# Autodesk Inventor assembly: #Spindexer
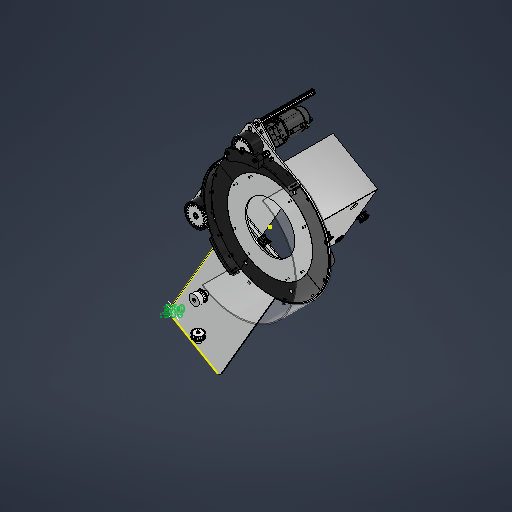
[picture p0: Inventor's stored thumbnail of the model, 512x512]
Saved by Autodesk Inventor 2026 (Build 300175000, 175)
## iProperties
Created: 2026-02-05
Part Number: #Spindexer
Document SubType Name: Assembly
Designer: Owen L
Mass: 7910.07 g
Surface Area: 22164.7 cm^2
Volume: 5901.9 cm^3
Density: 1.34026 g/cm^3
Author: Owen L
## Documents named in this file (54)
- C:\Users\littl\OneDrive\Documents\GitHub\2026-Robot-Mechanical\Spindexer\#Spindexer.iam
- C:\Users\littl\OneDrive\Documents\GitHub\2026-Robot-Mechanical\Spindexer\3DPRINT,KICKER,RAMP.ipt
- C:\Users\littl\OneDrive\Documents\GitHub\2026-Robot-Mechanical\#1_CAD Library\Power Transmission\Bearings\PURCHASED,HEX_BEARING.ipt
- C:\Users\littl\OneDrive\Documents\GitHub\2026-Robot-Mechanical\#1_CAD Library\Building Materials\Fasteners\Bolts\PURCHASED,10-32x0.5in,BUTTONHEAD,BOLT.ipt
- C:\Users\littl\OneDrive\Documents\GitHub\2026-Robot-Mechanical\#1_CAD Library\Building Materials\Fasteners\Nuts\PURCHASED,NYLOCK,10-32,NUT.ipt
- C:\Users\littl\OneDrive\Documents\GitHub\2026-Robot-Mechanical\#1_CAD Library\Building Materials\Fasteners\Bolts\PURCHASED,10-32x0.625in,BUTTONHEAD,BOLT.ipt
- C:\Users\littl\OneDrive\Documents\GitHub\2026-Robot-Mechanical\Spindexer\PLATE,SHOOTER,MOUNT.ipt
- C:\Users\littl\OneDrive\Documents\GitHub\2026-Robot-Mechanical\Spindexer\PLATE,TURRET,ENCODER,GEAR.ipt
- C:\Users\littl\OneDrive\Documents\GitHub\2026-Robot-Mechanical\Spindexer\PLATE,TURRET,PINNION,GEAR.ipt
- C:\Users\littl\OneDrive\Documents\GitHub\2026-Robot-Mechanical\Spindexer\PLATE,TURRET,MOTOR,MOUNT.ipt
- C:\Users\littl\OneDrive\Documents\GitHub\2026-Robot-Mechanical\#1_CAD Library\Electronics\CONTROLS,ENCODER,HEX_BORE.ipt
- C:\Users\littl\OneDrive\Documents\GitHub\2026-Robot-Mechanical\Spindexer\STOCK,HEX,SHAFT,TURRET,DRIVE.ipt
- C:\Users\littl\OneDrive\Documents\GitHub\2026-Robot-Mechanical\Spindexer\STOCK,HEX,SHAFT,TURRET,ENCODER.ipt
- C:\Users\littl\OneDrive\Documents\GitHub\2026-Robot-Mechanical\Spindexer\3DPRINT,TURRET,HEX,SPACER.ipt
- C:\Users\littl\OneDrive\Documents\GitHub\2026-Robot-Mechanical\Spindexer\STOCK,CHURRO,HEX,TURRET,MOTOR-MOUNT,SPACER.ipt
- C:\Users\littl\OneDrive\Documents\GitHub\2026-Robot-Mechanical\#1_CAD Library\Building Materials\Fasteners\Bolts\PURCHASED,0.25-20x0.5in,BUTTONHEAD,BOLT.ipt
- C:\Users\littl\OneDrive\Documents\GitHub\2026-Robot-Mechanical\Spindexer\MOTOR,VEX,FALCON,500.ipt
- C:\Users\littl\OneDrive\Documents\GitHub\2026-Robot-Mechanical\#1_CAD Library\Power Transmission\MaxPlanetary\PURCHASED,REV,MAX-PLANETARY,SINGLE-STAGE,FALCON-TO-HEX.ipt
- C:\Users\littl\OneDrive\Documents\GitHub\2026-Robot-Mechanical\#1_CAD Library\Building Materials\Fasteners\Washers\PURCHASED,WASHER,10-32.ipt
- C:\Users\littl\OneDrive\Documents\GitHub\2026-Robot-Mechanical\Spindexer\3DPRINT,CABLE-SHROUD,QUARTER.ipt
- C:\Users\littl\OneDrive\Documents\GitHub\2026-Robot-Mechanical\Spindexer\3DPRINT,CABLE,TRAY,BL.ipt
- C:\Users\littl\OneDrive\Documents\GitHub\2026-Robot-Mechanical\Spindexer\3DPRINT,CABLE,TRAY,BR.ipt
- C:\Users\littl\OneDrive\Documents\GitHub\2026-Robot-Mechanical\Spindexer\3DPRINT,CABLE,TRAY,TL.ipt
- C:\Users\littl\OneDrive\Documents\GitHub\2026-Robot-Mechanical\Spindexer\3DPRINT,CABLE,TRAY,TR.ipt
- C:\Users\littl\OneDrive\Documents\GitHub\2026-Robot-Mechanical\Spindexer\PLATE,SHOOTER,SHEILD,LOWER.ipt
- C:\Users\littl\OneDrive\Documents\GitHub\2026-Robot-Mechanical\Spindexer\3DPRINT,TURRET,PINION,SHROUD.ipt
- C:\Users\littl\OneDrive\Documents\GitHub\2026-Robot-Mechanical\#1_CAD Library\Building Materials\Fasteners\Bolts\PURCHASED,10-32x0.75in,BUTTONHEAD,BOLT.ipt
- C:\Users\littl\OneDrive\Documents\GitHub\2026-Robot-Mechanical\Spindexer\3DPRINT,TURRET,PINION,SHROUD,21T.ipt
- C:\Users\littl\OneDrive\Documents\GitHub\2026-Robot-Mechanical\Spindexer\STOCK,CHURRO,HEX,TURRET,MOTOR-MOUNT,SUPPORT.ipt
- C:\Users\littl\OneDrive\Documents\GitHub\2026-Robot-Mechanical\Spindexer\3DPRINT,TURRET,LOCK.ipt
- C:\Users\littl\OneDrive\Documents\GitHub\2026-Robot-Mechanical\Spindexer\STOCK,CHURRO,HEX,TURRET,LOCK.ipt
- C:\Users\littl\OneDrive\Documents\GitHub\2026-Robot-Mechanical\#1_CAD Library\Building Materials\Fasteners\Bolts\PURCHASED,0.25-20x0.875in,SOCKETHEAD,BOLT.ipt
- C:\Users\littl\OneDrive\Documents\GitHub\2026-Robot-Mechanical\Spindexer\PLATE,BACK.ipt
- C:\Users\littl\OneDrive\Documents\GitHub\2026-Robot-Mechanical\Spindexer\PLATE,FRONT.ipt
- C:\Users\littl\OneDrive\Documents\GitHub\2026-Robot-Mechanical\Spindexer\WCP-0564.ipt
- C:\Users\littl\OneDrive\Documents\GitHub\2026-Robot-Mechanical\#1_CAD Library\Wheels\Compliant\PURCHASED,WHEEL,COMPLIANT,2.25in.ipt
- C:\Users\littl\OneDrive\Documents\GitHub\2026-Robot-Mechanical\Spindexer\PLATE,BEARING,BLOCK.ipt
- C:\Users\littl\OneDrive\Documents\GitHub\2026-Robot-Mechanical\Spindexer\PLATE,BEARING,BLOCK,TOP.ipt
- C:\Users\littl\OneDrive\Documents\GitHub\2026-Robot-Mechanical\Spindexer\Kicker.ipt
- C:\Users\littl\OneDrive\Documents\GitHub\2026-Robot-Mechanical\#1_CAD Library\Motors\MOTOR,NEO,V2.0.ipt
- C:\Users\littl\OneDrive\Documents\GitHub\2026-Robot-Mechanical\Spindexer\PLATE_LEFT.ipt
- C:\Users\littl\OneDrive\Documents\GitHub\2026-Robot-Mechanical\Spindexer\PLATE,BELT,REVERSER.ipt
- C:\Users\littl\OneDrive\Documents\GitHub\2026-Robot-Mechanical\Spindexer\WCP-0562.ipt
- C:\Users\littl\OneDrive\Documents\GitHub\2026-Robot-Mechanical\Spindexer\REV-21-1921.ipt
- C:\Users\littl\OneDrive\Documents\GitHub\2026-Robot-Mechanical\Spindexer\WCP-2057.ipt
- C:\Users\littl\OneDrive\Documents\GitHub\2026-Robot-Mechanical\Spindexer\WCP-1420.ipt
- C:\Users\littl\OneDrive\Documents\GitHub\2026-Robot-Mechanical\Spindexer\STOCK,LEFT,HEX.ipt
- C:\Users\littl\OneDrive\Documents\GitHub\2026-Robot-Mechanical\Spindexer\STOCK,REVERSER,HEX.ipt
- C:\Users\littl\OneDrive\Documents\GitHub\2026-Robot-Mechanical\Spindexer\STOCK,TOP-RIGHT,HEX.ipt
- C:\Users\littl\OneDrive\Documents\GitHub\2026-Robot-Mechanical\Spindexer\STOCK,BOTTOM-RIGHT,HEX.ipt
- C:\Users\littl\OneDrive\Documents\GitHub\2026-Robot-Mechanical\Spindexer\3DPRINT,ROLLER,PLUG,SHORT.ipt
- C:\Users\littl\OneDrive\Documents\GitHub\2026-Robot-Mechanical\Spindexer\3DPRINT,ROLLER,PLUG,LONG.ipt
- C:\Users\littl\OneDrive\Documents\GitHub\2026-Robot-Mechanical\Spindexer\STOCK,KICKER,HEX.ipt
- C:\Users\littl\OneDrive\Documents\GitHub\2026-Robot-Mechanical\Spindexer\3DPRINT,VERTICAL,ROLLER,TOP,BEARING,BLOCK.ipt
## Components (129 placed, 53 different names)
1. 3DPRINT,VERTICAL,ROLLER,TOP,BEARING,BLOCK:1 — Mate:309, Insert:317
2. 3DPRINT,TURRET,PINION,SHROUD:1 — Mate:224, Mate:225, Mate:226, Insert:267
3. PURCHASED,10-32x0.75in,BUTTONHEAD,BOLT:1 — Insert:268, Mate:232
4. PURCHASED,10-32x0.75in,BUTTONHEAD,BOLT:2 — Insert:267, Mate:236
5. 3DPRINT,TURRET,PINION,SHROUD,21T:1 — Mate:227, Mate:228, Mate:229, Insert:268
6. STOCK,CHURRO,HEX,TURRET,MOTOR-MOUNT,SPACER:7 — Insert:272
7. STOCK,CHURRO,HEX,TURRET,MOTOR-MOUNT,SPACER:8 — Insert:273
8. PURCHASED,0.25-20x0.5in,BUTTONHEAD,BOLT:16 — Insert:279
9. PURCHASED,0.25-20x0.5in,BUTTONHEAD,BOLT:17 — Insert:280
10. PURCHASED,0.25-20x0.5in,BUTTONHEAD,BOLT:18 — Insert:281
11. STOCK,CHURRO,HEX,TURRET,MOTOR-MOUNT,SUPPORT:1 — Insert:282
12. 3DPRINT,TURRET,LOCK:1 — Mate:237, Mate:238, Flush:35, Insert:285, Insert:286
13. STOCK,CHURRO,HEX,TURRET,LOCK:1 — Insert:283
14. STOCK,CHURRO,HEX,TURRET,LOCK:2 — Insert:284
15. PURCHASED,0.25-20x0.875in,SOCKETHEAD,BOLT:1 — Insert:285
16. PURCHASED,0.25-20x0.875in,SOCKETHEAD,BOLT:2 — Insert:286
17. PURCHASED,0.25-20x0.5in,BUTTONHEAD,BOLT:19 — Insert:287
18. PURCHASED,0.25-20x0.5in,BUTTONHEAD,BOLT:20 — Insert:288
19. PLATE,BACK:1 — Mate:240, Mate:264, Flush:44, Mate:267, Flush:48, Flush:52, Mate:277, Mate:278, Mate:280, Insert:305, Insert:306, Insert:309, Insert:312, Insert:314, Insert:316, Mate:269
20. PLATE,FRONT:1 — Mate:264, Flush:44, Mate:265, Mate:268, Mate:270, Insert:303, Flush:49, Mate:274, Flush:51, Insert:311, Insert:313, Insert:315, Mate:306, Mate:311
21. WCP-0564:1 — Mate:267, Mate:298, Flush:64, Flush:66
22. PURCHASED,WHEEL,COMPLIANT,2.25in:1 — Mate:268, Mate:269, Insert:298, Mate:270
23. PURCHASED,WHEEL,COMPLIANT,2.25in:3 — Insert:298, Mate:309
24. PLATE,BEARING,BLOCK:1 — Flush:48, Flush:53, Insert:308
25. PLATE,BEARING,BLOCK,TOP:1 — Mate:272, Mate:278, Flush:53, Insert:310
26. KICKER_GEARBOX — Insert:303, Flush:49, Insert:304, Flush:50
27. MOTOR,NEO,V2.0:1 — Insert:304, Flush:50
28. PLATE_LEFT:1 — Mate:274, Flush:51, Mate:275
29. PLATE,BELT,REVERSER:1 — Mate:280, Insert:307
30. WCP-0562:1 — Mate:285, Flush:56, Flush:58
31. REV-21-1921:1 — Mate:282, Flush:54
32. REV-21-1921:2 — Mate:281, Flush:54, Mate:290, Mate:291
33. WCP-2057:1 — Insert:308, Mate:287, Flush:59
34. WCP-2057:2 — Insert:307, Mate:283, Mate:291, Flush:60
35. WCP-2057:3 — Insert:306, Mate:282, Mate:287, Mate:292, Mate:296
36. WCP-2057:4 — Insert:305, Mate:281, Mate:288, Mate:289, Mate:297
37. WCP-2057:5 — Insert:311, Flush:62
38. WCP-2057:6 — Insert:310, Mate:286, Flush:61
39. WCP-2057:7 — Insert:313, Flush:63
40. WCP-2057:8 — Insert:309, Mate:284, Mate:285, Mate:286, Mate:295
41. WCP-2057:9 — Insert:312, Mate:293, Mate:299, Mate:312
42. WCP-2057:11 — Insert:314, Mate:294, Mate:300
43. WCP-2057:12 — Insert:316, Mate:298
44. WCP-2057:13 — Insert:315, Mate:301, Mate:302, Mate:305
45. WCP-1420:1 — Mate:283, Mate:288, Flush:55, Mate:289, Mate:290
46. WCP-1420:2 — Mate:284, Flush:55
47. WCP-0562:2 — Mate:292, Flush:56
48. WCP-0562:3 — Mate:293, Flush:57, Flush:58
49. WCP-0562:4 — Mate:294, Flush:57
50. STOCK,LEFT,HEX:1 — Mate:295, Flush:61
51. STOCK,LEFT,HEX:2 — Mate:296, Flush:59
52. STOCK,REVERSER,HEX:1 — Mate:297, Flush:60
53. STOCK,TOP-RIGHT,HEX:1 — Mate:299, Flush:62
54. STOCK,BOTTOM-RIGHT,HEX:1 — Mate:300, Flush:63
55. 3DPRINT,ROLLER,PLUG,SHORT:1
56. 3DPRINT,ROLLER,PLUG,LONG:1
57. STOCK,KICKER,HEX:1 — Mate:301, Flush:64
58. WCP-1420:3 — Mate:302, Flush:65, Mate:310
59. WCP-1420:5 — Mate:305, Mate:310, Mate:311
60. WCP-1420:6
61. WCP-1420:7 — Mate:306, Flush:65
62. WCP-2057:14 — Insert:317
63. WCP-1420:8 — Mate:312, Flush:66
64. PURCHASED,10-32x0.625in,BUTTONHEAD,BOLT:45 — Insert:233
65. PURCHASED,NYLOCK,10-32,NUT:5 — Insert:234
66. PURCHASED,NYLOCK,10-32,NUT:6 — Insert:232
67. PURCHASED,0.25-20x0.5in,BUTTONHEAD,BOLT:9 — Insert:163
68. PURCHASED,0.25-20x0.5in,BUTTONHEAD,BOLT:8 — Insert:162
69. PURCHASED,0.25-20x0.5in,BUTTONHEAD,BOLT:6 — Insert:159
70. PURCHASED,0.25-20x0.5in,BUTTONHEAD,BOLT:5 — Insert:270
71. PURCHASED,NYLOCK,10-32,NUT:8 — Insert:236
72. PURCHASED,NYLOCK,10-32,NUT:7 — Insert:238
73. PURCHASED,10-32x0.625in,BUTTONHEAD,BOLT:47 — Insert:235
74. PURCHASED,0.25-20x0.5in,BUTTONHEAD,BOLT:4 — Insert:158
75. PURCHASED,10-32x0.625in,BUTTONHEAD,BOLT:61 — Insert:174
76. PURCHASED,10-32x0.625in,BUTTONHEAD,BOLT:60 — Insert:175
77. PURCHASED,10-32x0.625in,BUTTONHEAD,BOLT:59 — Insert:176
78. PURCHASED,10-32x0.625in,BUTTONHEAD,BOLT:58 — Insert:177
79. PURCHASED,0.25-20x0.5in,BUTTONHEAD,BOLT:15 — Insert:277
80. PURCHASED,0.25-20x0.5in,BUTTONHEAD,BOLT:14 — Insert:278
81. PURCHASED,0.25-20x0.5in,BUTTONHEAD,BOLT:13
82. PURCHASED,0.25-20x0.5in,BUTTONHEAD,BOLT:12 — Insert:276
83. PURCHASED,0.25-20x0.5in,BUTTONHEAD,BOLT:11 — Insert:169
84. PURCHASED,0.25-20x0.5in,BUTTONHEAD,BOLT:10 — Insert:168
85. PURCHASED,WASHER,10-32:11 — Insert:215, Insert:218
86. PURCHASED,WASHER,10-32:12 — Insert:217, Insert:220
87. PURCHASED,WASHER,10-32:13 — Insert:216, Insert:219
88. PURCHASED,10-32x0.625in,BUTTONHEAD,BOLT:62 — Insert:218
89. PURCHASED,10-32x0.625in,BUTTONHEAD,BOLT:63 — Insert:219
90. PURCHASED,10-32x0.625in,BUTTONHEAD,BOLT:64 — Insert:220
91. PURCHASED,10-32x0.5in,BUTTONHEAD,BOLT:11 — Insert:221
92. PURCHASED,10-32x0.5in,BUTTONHEAD,BOLT:13 — Insert:223
93. PURCHASED,10-32x0.5in,BUTTONHEAD,BOLT:12 — Insert:222
94. PURCHASED,10-32x0.5in,BUTTONHEAD,BOLT:14 — Insert:224
95. PURCHASED,10-32x0.5in,BUTTONHEAD,BOLT:15 — Insert:225
96. PURCHASED,10-32x0.5in,BUTTONHEAD,BOLT:16 — Insert:226
97. PURCHASED,10-32x0.5in,BUTTONHEAD,BOLT:17 — Insert:227
98. PURCHASED,10-32x0.5in,BUTTONHEAD,BOLT:18 — Insert:228
99. 3DPRINT,TURRET,HEX,SPACER:1 — Mate:94, Mate:102, Mate:144, Mate:145
100. 3DPRINT,TURRET,HEX,SPACER:2 — Mate:93, Mate:141, Mate:142
101. 3DPRINT,KICKER,RAMP:1 — Flush:52, Mate:277
102. 3DPRINT,CABLE,TRAY,TR:1 — Mate:219, Mate:220
103. 3DPRINT,CABLE,TRAY,TL:1 — Mate:217, Mate:218, Mate:219, Mate:220
104. 3DPRINT,CABLE,TRAY,BR:1 — Mate:215, Mate:216, Mate:217, Mate:218
105. 3DPRINT,CABLE,TRAY,BL:1 — Mate:213, Mate:214, Flush:33, Mate:215, Mate:216
106. 3DPRINT,CABLE-SHROUD,QUARTER:2 — Mate:205, Mate:206, Mate:207, Mate:223, Mate:226
107. 3DPRINT,CABLE-SHROUD,QUARTER:1 — Mate:202, Mate:203, Mate:204, Mate:205, Mate:207, Flush:33, Mate:228
108. PLATE,SHOOTER,MOUNT:1 — Mate:82, Mate:95, Mate:100, Insert:150, Insert:152, Insert:153, Insert:154, Insert:158, Insert:159, Insert:165, Insert:166, Insert:168, Insert:169, Insert:221, Insert:222, Insert:223, Insert:224, Insert:225, Insert:226, Insert:227, Insert:228, Insert:233, Insert:235, Mate:202, Mate:203, Mate:204, Mate:206, Mate:213, Mate:214, Mate:222, Flush:34, Mate:225, Mate:229, Mate:231, Insert:270, Mate:233, Mate:234, Mate:235, Insert:274, Insert:276, Insert:280, Insert:281, Mate:237, Mate:238, Insert:283, Insert:284, Insert:287, Insert:288, Mate:240, Mate:265, Mate:272, Mate:275
109. PLATE,TURRET,MOTOR,MOUNT:1 — Mate:100, Insert:155, Insert:157, Insert:162, Insert:163, Insert:174, Insert:175, Insert:176, Insert:177, Mate:147, Insert:178, Mate:148, Mate:231, Insert:269, Insert:282
110. PLATE,TURRET,MOTOR,MOUNT:2 — Mate:233, Mate:234, Mate:235, Insert:271, Insert:272, Insert:273, Insert:275, Insert:277, Insert:278, Insert:279
111. PLATE,TURRET,ENCODER,GEAR:1 — Mate:102, Mate:143, Flush:26
112. PLATE,TURRET,PINNION,GEAR:1 — Mate:86, Flush:25, Mate:140, Mate:141, Flush:35
113. PLATE,SHOOTER,SHEILD,LOWER:1 — Mate:222, Flush:34, Mate:223
114. STOCK,CHURRO,HEX,TURRET,MOTOR-MOUNT,SPACER:5 — Insert:165
115. STOCK,CHURRO,HEX,TURRET,MOTOR-MOUNT,SPACER:6 — Insert:166
116. STOCK,CHURRO,HEX,TURRET,MOTOR-MOUNT,SPACER:4 — Insert:271, Insert:274
117. STOCK,CHURRO,HEX,TURRET,MOTOR-MOUNT,SPACER:3 — Insert:269
118. STOCK,CHURRO,HEX,TURRET,MOTOR-MOUNT,SPACER:2 — Insert:152, Insert:157
119. STOCK,CHURRO,HEX,TURRET,MOTOR-MOUNT,SPACER:1 — Insert:150
120. STOCK,HEX,SHAFT,TURRET,ENCODER:1 — Mate:143, Flush:26, Mate:144, Insert:216, Insert:217, Mate:224
121. STOCK,HEX,SHAFT,TURRET,DRIVE:1 — Flush:25, Mate:140, Mate:142, Insert:215, Mate:227
122. PURCHASED,HEX_BEARING:6 — Mate:83, Mate:86, Mate:93, Insert:154
123. PURCHASED,HEX_BEARING:7 — Mate:94, Mate:96, Insert:153, Mate:145
124. CONTROLS,ENCODER,HEX_BORE:1 — Mate:95, Mate:96, Insert:236, Insert:238, Mate:236
125. CONTROLS,ENCODER,HEX_BORE:2 — Mate:82, Mate:83, Insert:232, Insert:234, Mate:232
126. PURCHASED,HEX_BEARING:8 — Insert:155
127. MOTOR,VEX,FALCON,500:1 — Insert:179, Mate:149
128. PURCHASED,REV,MAX-PLANETARY,SINGLE-STAGE,FALCON-TO-HEX:1 — Mate:147, Insert:178, Mate:148, Insert:179, Mate:149
129. PURCHASED,HEX_BEARING:9 — Insert:275
## Relationships (194: Mate 91, Insert 78, Flush 25)
- Mate:82: PLATE,SHOOTER,MOUNT:1 ↔ CONTROLS,ENCODER,HEX_BORE:2
- Mate:83: PURCHASED,HEX_BEARING:6 ↔ CONTROLS,ENCODER,HEX_BORE:2
- Mate:86: PLATE,TURRET,PINNION,GEAR:1 ↔ PURCHASED,HEX_BEARING:6
- Mate:93: 3DPRINT,TURRET,HEX,SPACER:2 ↔ PURCHASED,HEX_BEARING:6
- Mate:94: 3DPRINT,TURRET,HEX,SPACER:1 ↔ PURCHASED,HEX_BEARING:7
- Mate:95: PLATE,SHOOTER,MOUNT:1 ↔ CONTROLS,ENCODER,HEX_BORE:1
- Mate:96: PURCHASED,HEX_BEARING:7 ↔ CONTROLS,ENCODER,HEX_BORE:1
- Mate:100 (19.05 mm): PLATE,SHOOTER,MOUNT:1 ↔ PLATE,TURRET,MOTOR,MOUNT:1
- Mate:102: 3DPRINT,TURRET,HEX,SPACER:1 ↔ PLATE,TURRET,ENCODER,GEAR:1
- Insert:150: PLATE,SHOOTER,MOUNT:1 ↔ STOCK,CHURRO,HEX,TURRET,MOTOR-MOUNT,SPACER:1
- Insert:152: PLATE,SHOOTER,MOUNT:1 ↔ STOCK,CHURRO,HEX,TURRET,MOTOR-MOUNT,SPACER:2
- Insert:153: PLATE,SHOOTER,MOUNT:1 ↔ PURCHASED,HEX_BEARING:7
- Insert:154: PLATE,SHOOTER,MOUNT:1 ↔ PURCHASED,HEX_BEARING:6
- Insert:155: PLATE,TURRET,MOTOR,MOUNT:1 ↔ PURCHASED,HEX_BEARING:8
- Insert:157: PLATE,TURRET,MOTOR,MOUNT:1 ↔ STOCK,CHURRO,HEX,TURRET,MOTOR-MOUNT,SPACER:2
- Insert:158: PURCHASED,0.25-20x0.5in,BUTTONHEAD,BOLT:4 ↔ PLATE,SHOOTER,MOUNT:1
- Insert:159: PURCHASED,0.25-20x0.5in,BUTTONHEAD,BOLT:6 ↔ PLATE,SHOOTER,MOUNT:1
- Insert:162: PURCHASED,0.25-20x0.5in,BUTTONHEAD,BOLT:8 ↔ PLATE,TURRET,MOTOR,MOUNT:1
- Insert:163: PURCHASED,0.25-20x0.5in,BUTTONHEAD,BOLT:9 ↔ PLATE,TURRET,MOTOR,MOUNT:1
- Flush:25: PLATE,TURRET,PINNION,GEAR:1 ↔ STOCK,HEX,SHAFT,TURRET,DRIVE:1
- Mate:140: PLATE,TURRET,PINNION,GEAR:1 ↔ STOCK,HEX,SHAFT,TURRET,DRIVE:1
- Mate:141: 3DPRINT,TURRET,HEX,SPACER:2 ↔ PLATE,TURRET,PINNION,GEAR:1
- Mate:142: 3DPRINT,TURRET,HEX,SPACER:2 ↔ STOCK,HEX,SHAFT,TURRET,DRIVE:1
- Mate:143: PLATE,TURRET,ENCODER,GEAR:1 ↔ STOCK,HEX,SHAFT,TURRET,ENCODER:1
- Flush:26: PLATE,TURRET,ENCODER,GEAR:1 ↔ STOCK,HEX,SHAFT,TURRET,ENCODER:1
- Mate:144: 3DPRINT,TURRET,HEX,SPACER:1 ↔ STOCK,HEX,SHAFT,TURRET,ENCODER:1
- Mate:145: 3DPRINT,TURRET,HEX,SPACER:1 ↔ PURCHASED,HEX_BEARING:7
- Insert:165: PLATE,SHOOTER,MOUNT:1 ↔ STOCK,CHURRO,HEX,TURRET,MOTOR-MOUNT,SPACER:5
- Insert:166: PLATE,SHOOTER,MOUNT:1 ↔ STOCK,CHURRO,HEX,TURRET,MOTOR-MOUNT,SPACER:6
- Insert:168: PURCHASED,0.25-20x0.5in,BUTTONHEAD,BOLT:10 ↔ PLATE,SHOOTER,MOUNT:1
- Insert:169: PURCHASED,0.25-20x0.5in,BUTTONHEAD,BOLT:11 ↔ PLATE,SHOOTER,MOUNT:1
- Insert:174: PURCHASED,10-32x0.625in,BUTTONHEAD,BOLT:61 ↔ PLATE,TURRET,MOTOR,MOUNT:1
- Insert:175: PURCHASED,10-32x0.625in,BUTTONHEAD,BOLT:60 ↔ PLATE,TURRET,MOTOR,MOUNT:1
- Insert:176: PURCHASED,10-32x0.625in,BUTTONHEAD,BOLT:59 ↔ PLATE,TURRET,MOTOR,MOUNT:1
- Insert:177: PURCHASED,10-32x0.625in,BUTTONHEAD,BOLT:58 ↔ PLATE,TURRET,MOTOR,MOUNT:1
- Mate:147: PLATE,TURRET,MOTOR,MOUNT:1 ↔ PURCHASED,REV,MAX-PLANETARY,SINGLE-STAGE,FALCON-TO-HEX:1
- Insert:178: PLATE,TURRET,MOTOR,MOUNT:1 ↔ PURCHASED,REV,MAX-PLANETARY,SINGLE-STAGE,FALCON-TO-HEX:1
- Mate:148: PLATE,TURRET,MOTOR,MOUNT:1 ↔ PURCHASED,REV,MAX-PLANETARY,SINGLE-STAGE,FALCON-TO-HEX:1
- Insert:179: MOTOR,VEX,FALCON,500:1 ↔ PURCHASED,REV,MAX-PLANETARY,SINGLE-STAGE,FALCON-TO-HEX:1
- Mate:149: MOTOR,VEX,FALCON,500:1 ↔ PURCHASED,REV,MAX-PLANETARY,SINGLE-STAGE,FALCON-TO-HEX:1
- Insert:215: PURCHASED,WASHER,10-32:11 ↔ STOCK,HEX,SHAFT,TURRET,DRIVE:1
- Insert:216: PURCHASED,WASHER,10-32:13 ↔ STOCK,HEX,SHAFT,TURRET,ENCODER:1
- Insert:217: PURCHASED,WASHER,10-32:12 ↔ STOCK,HEX,SHAFT,TURRET,ENCODER:1
- Insert:218: PURCHASED,WASHER,10-32:11 ↔ PURCHASED,10-32x0.625in,BUTTONHEAD,BOLT:62
- Insert:219: PURCHASED,WASHER,10-32:13 ↔ PURCHASED,10-32x0.625in,BUTTONHEAD,BOLT:63
- Insert:220: PURCHASED,WASHER,10-32:12 ↔ PURCHASED,10-32x0.625in,BUTTONHEAD,BOLT:64
- Insert:221: PURCHASED,10-32x0.5in,BUTTONHEAD,BOLT:11 ↔ PLATE,SHOOTER,MOUNT:1
- Insert:222: PURCHASED,10-32x0.5in,BUTTONHEAD,BOLT:12 ↔ PLATE,SHOOTER,MOUNT:1
- Insert:223: PURCHASED,10-32x0.5in,BUTTONHEAD,BOLT:13 ↔ PLATE,SHOOTER,MOUNT:1
- Insert:224: PURCHASED,10-32x0.5in,BUTTONHEAD,BOLT:14 ↔ PLATE,SHOOTER,MOUNT:1
- Insert:225: PURCHASED,10-32x0.5in,BUTTONHEAD,BOLT:15 ↔ PLATE,SHOOTER,MOUNT:1
- Insert:226: PURCHASED,10-32x0.5in,BUTTONHEAD,BOLT:16 ↔ PLATE,SHOOTER,MOUNT:1
- Insert:227: PURCHASED,10-32x0.5in,BUTTONHEAD,BOLT:17 ↔ PLATE,SHOOTER,MOUNT:1
- Insert:228: PURCHASED,10-32x0.5in,BUTTONHEAD,BOLT:18 ↔ PLATE,SHOOTER,MOUNT:1
- Insert:232: PURCHASED,NYLOCK,10-32,NUT:6 ↔ CONTROLS,ENCODER,HEX_BORE:2
- Insert:233: PURCHASED,10-32x0.625in,BUTTONHEAD,BOLT:45 ↔ PLATE,SHOOTER,MOUNT:1
- Insert:234: PURCHASED,NYLOCK,10-32,NUT:5 ↔ CONTROLS,ENCODER,HEX_BORE:2
- Insert:235: PURCHASED,10-32x0.625in,BUTTONHEAD,BOLT:47 ↔ PLATE,SHOOTER,MOUNT:1
- Insert:236: PURCHASED,NYLOCK,10-32,NUT:8 ↔ CONTROLS,ENCODER,HEX_BORE:1
- Insert:238: PURCHASED,NYLOCK,10-32,NUT:7 ↔ CONTROLS,ENCODER,HEX_BORE:1
- Mate:202: 3DPRINT,CABLE-SHROUD,QUARTER:1 ↔ PLATE,SHOOTER,MOUNT:1
- Mate:203: 3DPRINT,CABLE-SHROUD,QUARTER:1 ↔ PLATE,SHOOTER,MOUNT:1
- Mate:204: 3DPRINT,CABLE-SHROUD,QUARTER:1 ↔ PLATE,SHOOTER,MOUNT:1
- Mate:205: 3DPRINT,CABLE-SHROUD,QUARTER:2 ↔ 3DPRINT,CABLE-SHROUD,QUARTER:1
- Mate:206: 3DPRINT,CABLE-SHROUD,QUARTER:2 ↔ PLATE,SHOOTER,MOUNT:1
- Mate:207: 3DPRINT,CABLE-SHROUD,QUARTER:2 ↔ 3DPRINT,CABLE-SHROUD,QUARTER:1
- Mate:213: 3DPRINT,CABLE,TRAY,BL:1 ↔ PLATE,SHOOTER,MOUNT:1
- Mate:214: 3DPRINT,CABLE,TRAY,BL:1 ↔ PLATE,SHOOTER,MOUNT:1
- Flush:33: 3DPRINT,CABLE,TRAY,BL:1 ↔ 3DPRINT,CABLE-SHROUD,QUARTER:1
- Mate:215: 3DPRINT,CABLE,TRAY,BR:1 ↔ 3DPRINT,CABLE,TRAY,BL:1
- Mate:216: 3DPRINT,CABLE,TRAY,BR:1 ↔ 3DPRINT,CABLE,TRAY,BL:1
- Mate:217: 3DPRINT,CABLE,TRAY,TL:1 ↔ 3DPRINT,CABLE,TRAY,BR:1
- Mate:218: 3DPRINT,CABLE,TRAY,TL:1 ↔ 3DPRINT,CABLE,TRAY,BR:1
- Mate:219: 3DPRINT,CABLE,TRAY,TR:1 ↔ 3DPRINT,CABLE,TRAY,TL:1
- Mate:220: 3DPRINT,CABLE,TRAY,TR:1 ↔ 3DPRINT,CABLE,TRAY,TL:1
- Mate:222: PLATE,SHOOTER,MOUNT:1 ↔ PLATE,SHOOTER,SHEILD,LOWER:1
- Flush:34: PLATE,SHOOTER,MOUNT:1 ↔ PLATE,SHOOTER,SHEILD,LOWER:1
- Mate:223: 3DPRINT,CABLE-SHROUD,QUARTER:2 ↔ PLATE,SHOOTER,SHEILD,LOWER:1
- Mate:224: 3DPRINT,TURRET,PINION,SHROUD:1 ↔ STOCK,HEX,SHAFT,TURRET,ENCODER:1
- Mate:225: 3DPRINT,TURRET,PINION,SHROUD:1 ↔ PLATE,SHOOTER,MOUNT:1
- Mate:226: 3DPRINT,TURRET,PINION,SHROUD:1 ↔ 3DPRINT,CABLE-SHROUD,QUARTER:2
- Insert:267: 3DPRINT,TURRET,PINION,SHROUD:1 ↔ PURCHASED,10-32x0.75in,BUTTONHEAD,BOLT:2
- Mate:227: 3DPRINT,TURRET,PINION,SHROUD,21T:1 ↔ STOCK,HEX,SHAFT,TURRET,DRIVE:1
- Mate:228: 3DPRINT,TURRET,PINION,SHROUD,21T:1 ↔ 3DPRINT,CABLE-SHROUD,QUARTER:1
- Mate:229: 3DPRINT,TURRET,PINION,SHROUD,21T:1 ↔ PLATE,SHOOTER,MOUNT:1
- Insert:268: PURCHASED,10-32x0.75in,BUTTONHEAD,BOLT:1 ↔ 3DPRINT,TURRET,PINION,SHROUD,21T:1
- Mate:231: PLATE,SHOOTER,MOUNT:1 ↔ PLATE,TURRET,MOTOR,MOUNT:1
- Insert:269: PLATE,TURRET,MOTOR,MOUNT:1 ↔ STOCK,CHURRO,HEX,TURRET,MOTOR-MOUNT,SPACER:3
- Insert:270: PURCHASED,0.25-20x0.5in,BUTTONHEAD,BOLT:5 ↔ PLATE,SHOOTER,MOUNT:1
- Mate:232: PURCHASED,10-32x0.75in,BUTTONHEAD,BOLT:1 ↔ CONTROLS,ENCODER,HEX_BORE:2
- Mate:233: PLATE,SHOOTER,MOUNT:1 ↔ PLATE,TURRET,MOTOR,MOUNT:2
- Mate:234: PLATE,SHOOTER,MOUNT:1 ↔ PLATE,TURRET,MOTOR,MOUNT:2
- Mate:235: PLATE,SHOOTER,MOUNT:1 ↔ PLATE,TURRET,MOTOR,MOUNT:2
- Insert:271: PLATE,TURRET,MOTOR,MOUNT:2 ↔ STOCK,CHURRO,HEX,TURRET,MOTOR-MOUNT,SPACER:4
- Insert:272: STOCK,CHURRO,HEX,TURRET,MOTOR-MOUNT,SPACER:7 ↔ PLATE,TURRET,MOTOR,MOUNT:2
- Insert:273: STOCK,CHURRO,HEX,TURRET,MOTOR-MOUNT,SPACER:8 ↔ PLATE,TURRET,MOTOR,MOUNT:2
- Insert:274: PLATE,SHOOTER,MOUNT:1 ↔ STOCK,CHURRO,HEX,TURRET,MOTOR-MOUNT,SPACER:4
- Insert:275: PLATE,TURRET,MOTOR,MOUNT:2 ↔ PURCHASED,HEX_BEARING:9
- Insert:276: PURCHASED,0.25-20x0.5in,BUTTONHEAD,BOLT:12 ↔ PLATE,SHOOTER,MOUNT:1
- Insert:277: PURCHASED,0.25-20x0.5in,BUTTONHEAD,BOLT:15 ↔ PLATE,TURRET,MOTOR,MOUNT:2
- Insert:278: PURCHASED,0.25-20x0.5in,BUTTONHEAD,BOLT:14 ↔ PLATE,TURRET,MOTOR,MOUNT:2
- Mate:236: PURCHASED,10-32x0.75in,BUTTONHEAD,BOLT:2 ↔ CONTROLS,ENCODER,HEX_BORE:1
- Insert:279: PURCHASED,0.25-20x0.5in,BUTTONHEAD,BOLT:16 ↔ PLATE,TURRET,MOTOR,MOUNT:2
- Insert:280: PURCHASED,0.25-20x0.5in,BUTTONHEAD,BOLT:17 ↔ PLATE,SHOOTER,MOUNT:1
- Insert:281: PURCHASED,0.25-20x0.5in,BUTTONHEAD,BOLT:18 ↔ PLATE,SHOOTER,MOUNT:1
- Insert:282: STOCK,CHURRO,HEX,TURRET,MOTOR-MOUNT,SUPPORT:1 ↔ PLATE,TURRET,MOTOR,MOUNT:1
- Mate:237: 3DPRINT,TURRET,LOCK:1 ↔ PLATE,SHOOTER,MOUNT:1
- Mate:238: 3DPRINT,TURRET,LOCK:1 ↔ PLATE,SHOOTER,MOUNT:1
- Flush:35: 3DPRINT,TURRET,LOCK:1 ↔ PLATE,TURRET,PINNION,GEAR:1
- Insert:283: STOCK,CHURRO,HEX,TURRET,LOCK:1 ↔ PLATE,SHOOTER,MOUNT:1
- Insert:284: STOCK,CHURRO,HEX,TURRET,LOCK:2 ↔ PLATE,SHOOTER,MOUNT:1
- Insert:285: 3DPRINT,TURRET,LOCK:1 ↔ PURCHASED,0.25-20x0.875in,SOCKETHEAD,BOLT:1
- Insert:286: 3DPRINT,TURRET,LOCK:1 ↔ PURCHASED,0.25-20x0.875in,SOCKETHEAD,BOLT:2
- Insert:287: PURCHASED,0.25-20x0.5in,BUTTONHEAD,BOLT:19 ↔ PLATE,SHOOTER,MOUNT:1
- Insert:288: PURCHASED,0.25-20x0.5in,BUTTONHEAD,BOLT:20 ↔ PLATE,SHOOTER,MOUNT:1
- Mate:240: PLATE,BACK:1 ↔ PLATE,SHOOTER,MOUNT:1
- Mate:264 (158.75 mm): PLATE,BACK:1 ↔ PLATE,FRONT:1
- Flush:44: PLATE,BACK:1 ↔ PLATE,FRONT:1
- Mate:265: PLATE,FRONT:1 ↔ PLATE,SHOOTER,MOUNT:1
- Mate:267: PLATE,BACK:1 ↔ WCP-0564:1
- Mate:268 (-208.788 mm): PLATE,FRONT:1 ↔ PURCHASED,WHEEL,COMPLIANT,2.25in:1
- Mate:269 (179.832 mm): PLATE,BACK:1 ↔ PURCHASED,WHEEL,COMPLIANT,2.25in:1
- Insert:298: PURCHASED,WHEEL,COMPLIANT,2.25in:1 ↔ PURCHASED,WHEEL,COMPLIANT,2.25in:3
- Mate:270 (6.35 mm): PLATE,FRONT:1 ↔ PURCHASED,WHEEL,COMPLIANT,2.25in:1
- Mate:272: PLATE,BEARING,BLOCK,TOP:1 ↔ PLATE,SHOOTER,MOUNT:1
- Flush:48: PLATE,BACK:1 ↔ PLATE,BEARING,BLOCK:1
- Insert:303: PLATE,FRONT:1 ↔ KICKER_GEARBOX
- Flush:49: PLATE,FRONT:1 ↔ KICKER_GEARBOX
- Insert:304: KICKER_GEARBOX ↔ MOTOR,NEO,V2.0:1
- Flush:50: KICKER_GEARBOX ↔ MOTOR,NEO,V2.0:1
- Mate:274: PLATE,FRONT:1 ↔ PLATE_LEFT:1
- Flush:51: PLATE,FRONT:1 ↔ PLATE_LEFT:1
- Mate:275: PLATE_LEFT:1 ↔ PLATE,SHOOTER,MOUNT:1
- Flush:52: PLATE,BACK:1 ↔ 3DPRINT,KICKER,RAMP:1
- Mate:277: PLATE,BACK:1 ↔ 3DPRINT,KICKER,RAMP:1
- Mate:278 (95.25 mm): PLATE,BACK:1 ↔ PLATE,BEARING,BLOCK,TOP:1
- Flush:53: PLATE,BEARING,BLOCK:1 ↔ PLATE,BEARING,BLOCK,TOP:1
- Mate:280: PLATE,BACK:1 ↔ PLATE,BELT,REVERSER:1
- Insert:305: PLATE,BACK:1 ↔ WCP-2057:4
- Insert:306: PLATE,BACK:1 ↔ WCP-2057:3
- Insert:307: PLATE,BELT,REVERSER:1 ↔ WCP-2057:2
- Insert:308: PLATE,BEARING,BLOCK:1 ↔ WCP-2057:1
- Insert:309: PLATE,BACK:1 ↔ WCP-2057:8
- Insert:310: PLATE,BEARING,BLOCK,TOP:1 ↔ WCP-2057:6
- Insert:311: PLATE,FRONT:1 ↔ WCP-2057:5
- Insert:312: PLATE,BACK:1 ↔ WCP-2057:9
- Insert:313: PLATE,FRONT:1 ↔ WCP-2057:7
- Insert:314: PLATE,BACK:1 ↔ WCP-2057:11
- Insert:315: PLATE,FRONT:1 ↔ WCP-2057:13
- Insert:316: PLATE,BACK:1 ↔ WCP-2057:12
- Mate:281: REV-21-1921:2 ↔ WCP-2057:4
- Mate:282: REV-21-1921:1 ↔ WCP-2057:3
- Flush:54: REV-21-1921:1 ↔ REV-21-1921:2
- Mate:283: WCP-2057:2 ↔ WCP-1420:1
- Mate:284: WCP-2057:8 ↔ WCP-1420:2
- Mate:285: WCP-0562:1 ↔ WCP-2057:8
- Mate:286: WCP-2057:6 ↔ WCP-2057:8
- Mate:287: WCP-2057:1 ↔ WCP-2057:3
- Mate:288: WCP-2057:4 ↔ WCP-1420:1
- Flush:55: WCP-1420:1 ↔ WCP-1420:2
- Mate:289: WCP-2057:4 ↔ WCP-1420:1
- Mate:290: REV-21-1921:2 ↔ WCP-1420:1
- Mate:291: REV-21-1921:2 ↔ WCP-2057:2
- Mate:292: WCP-2057:3 ↔ WCP-0562:2
- Mate:293: WCP-2057:9 ↔ WCP-0562:3
- Mate:294: WCP-2057:11 ↔ WCP-0562:4
- Flush:56: WCP-0562:1 ↔ WCP-0562:2
- Flush:57: WCP-0562:3 ↔ WCP-0562:4
- Flush:58: WCP-0562:1 ↔ WCP-0562:3
- Mate:295: WCP-2057:8 ↔ STOCK,LEFT,HEX:1
- Mate:296: WCP-2057:3 ↔ STOCK,LEFT,HEX:2
- Mate:297: WCP-2057:4 ↔ STOCK,REVERSER,HEX:1
- Mate:298: WCP-0564:1 ↔ WCP-2057:12
- Mate:299: WCP-2057:9 ↔ STOCK,TOP-RIGHT,HEX:1
- Mate:300: WCP-2057:11 ↔ STOCK,BOTTOM-RIGHT,HEX:1
- Flush:59: WCP-2057:1 ↔ STOCK,LEFT,HEX:2
- Flush:60: WCP-2057:2 ↔ STOCK,REVERSER,HEX:1
- Flush:61: WCP-2057:6 ↔ STOCK,LEFT,HEX:1
- Flush:62: WCP-2057:5 ↔ STOCK,TOP-RIGHT,HEX:1
- Flush:63: WCP-2057:7 ↔ STOCK,BOTTOM-RIGHT,HEX:1
- Mate:301: WCP-2057:13 ↔ STOCK,KICKER,HEX:1
- Flush:64: WCP-0564:1 ↔ STOCK,KICKER,HEX:1
- Mate:302: WCP-2057:13 ↔ WCP-1420:3
- Mate:305: WCP-2057:13 ↔ WCP-1420:5
- Mate:306: PLATE,FRONT:1 ↔ WCP-1420:7
- [Mate]: 3DPRINT,VERTICAL,ROLLER,TOP,BEARING,BLOCK:1 ↔ PURCHASED,WHEEL,COMPLIANT,2.25in:3
- [Mate]: 3DPRINT,VERTICAL,ROLLER,TOP,BEARING,BLOCK:1 ↔ PLATE,FRONT:1
- Mate:309 (12.7 mm): 3DPRINT,VERTICAL,ROLLER,TOP,BEARING,BLOCK:1 ↔ PURCHASED,WHEEL,COMPLIANT,2.25in:3
- Insert:317: 3DPRINT,VERTICAL,ROLLER,TOP,BEARING,BLOCK:1 ↔ WCP-2057:14
- Flush:65: WCP-1420:3 ↔ WCP-1420:7
- Mate:310: WCP-1420:3 ↔ WCP-1420:5
- Mate:311 (10.7632 mm): PLATE,FRONT:1 ↔ WCP-1420:5
- Mate:312: WCP-2057:9 ↔ WCP-1420:8
- Flush:66: WCP-0564:1 ↔ WCP-1420:8
